# Autodesk Inventor assembly: fixedMount
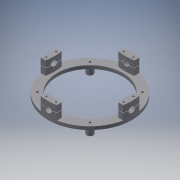
[picture p0: Inventor's stored thumbnail of the model, 180x180]
Saved by Autodesk Inventor 2016 SP1 (Build 200210100, 210)
## iProperties
Created: 2016-01-13
Part Number: fixedMount
Document SubType Name: Assembly
Designer: ddeboer
Author: ddeboer
## Documents named in this file (4)
- C:\Users\ddeboer\Desktop\leuschner-cad\fixedMount.iam
- C:\Users\ddeboer\Desktop\leuschner-cad\fixedRing.ipt
- C:\Users\ddeboer\Desktop\leuschner-cad\wedgeBlock.ipt
- C:\Users\ddeboer\Desktop\leuschner-cad\spacer.ipt
## Components (13 placed, 3 different names)
1. fixedRing:1 — Insert:1, Insert:2, Insert:4
2. wedgeBlock:1 — Insert:1, Insert:2, Insert:3, Flush:1
3. wedgeBlock:2
4. wedgeBlock:3
5. wedgeBlock:4
6. wedgeBlock:5 — Insert:3, Flush:1
7. wedgeBlock:6
8. wedgeBlock:7
9. wedgeBlock:8
10. spacer:1 — Insert:4
11. spacer:2
12. spacer:3
13. spacer:4
## Component patterns: (4 elements, first: wedgeBlock:1), (4 elements, first: wedgeBlock:5), (4 elements, first: spacer:1)
## Relationships (5: Insert 4, Flush 1)
- Insert:1: fixedRing:1 ↔ wedgeBlock:1
- Insert:2: fixedRing:1 ↔ wedgeBlock:1
- Insert:3 (1.524 mm): wedgeBlock:1 ↔ wedgeBlock:5
- Flush:1: wedgeBlock:1 ↔ wedgeBlock:5
- Insert:4: fixedRing:1 ↔ spacer:1
